# Autodesk Inventor assembly: POM_T5_23
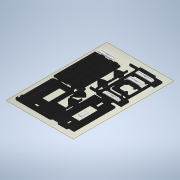
[picture p0: Inventor's stored thumbnail of the model, 180x180]
Saved by Autodesk Inventor 2020 (Build 240168000, 168)
## iProperties
Created: 2021-08-27
Part Number: POM_T5_23
Document SubType Name: Assembly
Designer: Masato
Author: Masato
## Documents named in this file (13)
- C:\Inventor\SUSTAINA-OP\Cam\POM_T5_23.iam
- C:\Inventor\SUSTAINA-OP\Cam\DisposableBoard.ipt
- C:\Inventor\SUSTAINA-OP\UpperBody\Cockpit\Cockpit_battery_bottom_frame.ipt
- C:\Inventor\SUSTAINA-OP\UpperBody\Cockpit\Cockpit_carrier_board_frame.ipt
- C:\Inventor\SUSTAINA-OP\UpperBody\Head\Camera_root_frame_e-CAM50_CUNX.ipt
- C:\Inventor\SUSTAINA-OP\UpperBody\Cockpit\Cockpit_side_frame_MIR.ipt
- C:\Inventor\SUSTAINA-OP\UpperBody\Cockpit\Cockpit_battery_front_frame.ipt
- C:\Inventor\SUSTAINA-OP\UpperBody\Cockpit\Cockpit_back_frame.ipt
- C:\Inventor\SUSTAINA-OP\UpperBody\Head\Camera_side_frame.ipt
- C:\Inventor\SUSTAINA-OP\Jig\Cockpit_battery_bottom_frame_Jig_2.ipt
- C:\Inventor\SUSTAINA-OP\Jig\Cockpit_battery_front_frame_Jig.ipt
- C:\Inventor\SUSTAINA-OP\Jig\Cockpit_battery_front_frame_Jig_2.ipt
- C:\Inventor\SUSTAINA-OP\Jig\Cockpit_side_frame_Jig.ipt
## Components (16 placed, 12 different names)
1. DisposableBoard:1 — メイト:2, メイト:1, フラッシュ:1, フラッシュ:2, メイト:4, メイト:5, メイト:6, メイト:7, フラッシュ:3, フラッシュ:4, フラッシュ:5, メイト:11, メイト:14, メイト:15, 角度:1, フラッシュ:8, メイト:19, メイト:21, メイト:28, メイト:31, メイト:33, メイト:36, メイト:40
2. Cockpit_side_frame_MIR:1 — メイト:4, フラッシュ:4, フラッシュ:5, メイト:10, メイト:12, フラッシュ:7, メイト:16, メイト:18
3. Cockpit_battery_bottom_frame:1 — メイト:5, フラッシュ:3, メイト:8, メイト:10, フラッシュ:6, フラッシュ:12
4. Cockpit_battery_front_frame:1 — メイト:6, メイト:8, フラッシュ:6, 正接:2
5. Cockpit_carrier_board_frame:1 — メイト:7, メイト:13, フラッシュ:8, メイト:20, メイト:22, メイト:23, メイト:29, メイト:30, メイト:34, メイト:35
6. Cockpit_back_frame:1 — メイト:11, メイト:12, フラッシュ:7, メイト:13, メイト:17, メイト:37, メイト:38
7. Camera_root_frame_e-CAM50_CUNX:1 — メイト:21, メイト:22, メイト:23, フラッシュ:11, メイト:32
8. Camera_side_frame:1 — メイト:14, メイト:16, メイト:17, 正接:1
9. Camera_side_frame:2 — メイト:15, 角度:1, 正接:1, メイト:18
10. Cockpit_battery_bottom_frame_Jig_2:1 — メイト:28, メイト:29, メイト:30
11. Cockpit_battery_front_frame_Jig:1 — メイト:31, フラッシュ:11, メイト:32
12. Cockpit_battery_front_frame_Jig_2:1 — メイト:33, メイト:34, メイト:35
13. Cockpit_side_frame_Jig:1 — メイト:36, メイト:37, メイト:38
14. Cockpit_battery_bottom_frame_Jig_2:2 — メイト:40, フラッシュ:12
15. Camera_side_frame:3 — メイト:19, メイト:20, 正接:2
16. Camera_side_frame:4
## Component patterns: (2 elements, first: Camera_side_frame:3)
## Relationships (46: Mate 33, Flush 10, Tangent 2, Angle 1)
- メイト:2 [Mate]: DisposableBoard:1
- メイト:1 [Mate]: DisposableBoard:1
- フラッシュ:1 [Flush]: DisposableBoard:1
- フラッシュ:2 [Flush]: DisposableBoard:1
- メイト:4 [Mate]: DisposableBoard:1 ↔ Cockpit_side_frame_MIR:1
- メイト:5 [Mate]: DisposableBoard:1 ↔ Cockpit_battery_bottom_frame:1
- メイト:6 [Mate]: DisposableBoard:1 ↔ Cockpit_battery_front_frame:1
- メイト:7 [Mate]: DisposableBoard:1 ↔ Cockpit_carrier_board_frame:1
- フラッシュ:3 [Flush] (2 mm): DisposableBoard:1 ↔ Cockpit_battery_bottom_frame:1
- メイト:8 [Mate] (2.5 mm): Cockpit_battery_bottom_frame:1 ↔ Cockpit_battery_front_frame:1
- フラッシュ:4 [Flush] (2 mm): DisposableBoard:1 ↔ Cockpit_side_frame_MIR:1
- フラッシュ:5 [Flush] (2 mm): DisposableBoard:1 ↔ Cockpit_side_frame_MIR:1
- メイト:10 [Mate] (2.5 mm): Cockpit_side_frame_MIR:1 ↔ Cockpit_battery_bottom_frame:1
- フラッシュ:6 [Flush] (2 mm): Cockpit_battery_bottom_frame:1 ↔ Cockpit_battery_front_frame:1
- メイト:11 [Mate]: DisposableBoard:1 ↔ Cockpit_back_frame:1
- メイト:12 [Mate] (2.5 mm): Cockpit_side_frame_MIR:1 ↔ Cockpit_back_frame:1
- フラッシュ:7 [Flush]: Cockpit_side_frame_MIR:1 ↔ Cockpit_back_frame:1
- メイト:13 [Mate] (2.5 mm): Cockpit_carrier_board_frame:1 ↔ Cockpit_back_frame:1
- メイト:14 [Mate]: DisposableBoard:1 ↔ Camera_side_frame:1
- メイト:15 [Mate]: DisposableBoard:1 ↔ Camera_side_frame:2
- メイト:16 [Mate] (2.5 mm): Cockpit_side_frame_MIR:1 ↔ Camera_side_frame:1
- メイト:17 [Mate] (2.5 mm): Cockpit_back_frame:1 ↔ Camera_side_frame:1
- 角度:1 [Angle] (270 deg): DisposableBoard:1 ↔ Camera_side_frame:2
- 正接:1 [Tangent] (2.5 mm): Camera_side_frame:1 ↔ Camera_side_frame:2
- メイト:18 [Mate] (2.5 mm): Cockpit_side_frame_MIR:1 ↔ Camera_side_frame:2
- フラッシュ:8 [Flush] (2.5 mm): DisposableBoard:1 ↔ Cockpit_carrier_board_frame:1
- メイト:19 [Mate]: DisposableBoard:1 ↔ Camera_side_frame:3
- メイト:20 [Mate] (2.5 mm): Cockpit_carrier_board_frame:1 ↔ Camera_side_frame:3
- 正接:2 [Tangent] (2.5 mm): Cockpit_battery_front_frame:1 ↔ Camera_side_frame:3
- メイト:21 [Mate]: DisposableBoard:1 ↔ Camera_root_frame_e-CAM50_CUNX:1
- メイト:22 [Mate] (9.5 mm): Cockpit_carrier_board_frame:1 ↔ Camera_root_frame_e-CAM50_CUNX:1
- メイト:23 [Mate] (5 mm): Cockpit_carrier_board_frame:1 ↔ Camera_root_frame_e-CAM50_CUNX:1
- メイト:28 [Mate]: DisposableBoard:1 ↔ Cockpit_battery_bottom_frame_Jig_2:1
- メイト:29 [Mate] (2.5 mm): Cockpit_carrier_board_frame:1 ↔ Cockpit_battery_bottom_frame_Jig_2:1
- メイト:30 [Mate] (2.5 mm): Cockpit_carrier_board_frame:1 ↔ Cockpit_battery_bottom_frame_Jig_2:1
- メイト:31 [Mate]: DisposableBoard:1 ↔ Cockpit_battery_front_frame_Jig:1
- フラッシュ:11 [Flush]: Camera_root_frame_e-CAM50_CUNX:1 ↔ Cockpit_battery_front_frame_Jig:1
- メイト:32 [Mate] (2.5 mm): Camera_root_frame_e-CAM50_CUNX:1 ↔ Cockpit_battery_front_frame_Jig:1
- メイト:33 [Mate]: DisposableBoard:1 ↔ Cockpit_battery_front_frame_Jig_2:1
- メイト:34 [Mate] (2.5 mm): Cockpit_carrier_board_frame:1 ↔ Cockpit_battery_front_frame_Jig_2:1
- メイト:35 [Mate] (8.5 mm): Cockpit_carrier_board_frame:1 ↔ Cockpit_battery_front_frame_Jig_2:1
- メイト:36 [Mate]: DisposableBoard:1 ↔ Cockpit_side_frame_Jig:1
- メイト:37 [Mate] (8.5 mm): Cockpit_back_frame:1 ↔ Cockpit_side_frame_Jig:1
- メイト:38 [Mate] (18.5 mm): Cockpit_back_frame:1 ↔ Cockpit_side_frame_Jig:1
- メイト:40 [Mate]: DisposableBoard:1 ↔ Cockpit_battery_bottom_frame_Jig_2:2
- フラッシュ:12 [Flush] (1 mm): Cockpit_battery_bottom_frame:1 ↔ Cockpit_battery_bottom_frame_Jig_2:2
